# Autodesk Inventor assembly: Prototype1
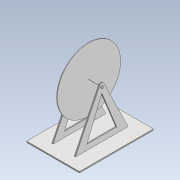
[picture p0: Inventor's stored thumbnail of the model, 180x180]
Saved by Autodesk Inventor 2021 (Build 250183000, 183)
## iProperties
Created: 2021-08-28
Part Number: Prototype1
Document SubType Name: Assembly
Designer: digge
Author: digge
## Documents named in this file (5)
- C:\Users\digge\Documents\Inventor\Projects\FerrisWheel\Prototype1.iam
- C:\Users\digge\Documents\Inventor\Projects\FerrisWheel\Base.ipt
- C:\Users\digge\Documents\Inventor\Projects\FerrisWheel\Stand.ipt
- C:\Users\digge\Documents\Inventor\Projects\FerrisWheel\Screw.ipt
- C:\Users\digge\Documents\Inventor\Projects\FerrisWheel\WheelFace.ipt
## Components (8 placed, 4 different names)
1. Base:1 — Flush:1, Mate:1, Flush:2, Mate:2, Mate:3, Mate:5, Mate:6, Mate:7, Mate:9
2. Stand:1 — Flush:4, Mate:4, Mate:5
3. Stand:2 — Flush:3, Mate:2, Mate:3, Mate:4, Insert:1
4. Stand:3 — Flush:5, Mate:6, Mate:7, Mate:8
5. Stand:4 — Flush:6, Mate:8, Mate:9
6. Base:2 — Flush:1, Mate:1, Flush:2, Flush:3, Flush:4, Flush:5, Flush:6
7. Screw:1 — Insert:1, Mate:10
8. WheelFace:1 — Mate:10
## Relationships (17: Mate 10, Flush 6, Insert 1)
- Flush:1: Base:1 ↔ Base:2
- Mate:1: Base:1 ↔ Base:2
- Flush:2: Base:1 ↔ Base:2
- Flush:3: Stand:2 ↔ Base:2
- Mate:2: Base:1 ↔ Stand:2
- Mate:3: Base:1 ↔ Stand:2
- Flush:4: Stand:1 ↔ Base:2
- Mate:4: Stand:1 ↔ Stand:2
- Mate:5: Base:1 ↔ Stand:1
- Flush:5: Stand:3 ↔ Base:2
- Mate:6: Base:1 ↔ Stand:3
- Mate:7: Base:1 ↔ Stand:3
- Flush:6: Stand:4 ↔ Base:2
- Mate:8: Stand:3 ↔ Stand:4
- Mate:9: Base:1 ↔ Stand:4
- Insert:1: Stand:2 ↔ Screw:1
- Mate:10: Screw:1 ↔ WheelFace:1
